# Autodesk Inventor assembly: Gearbox Handle
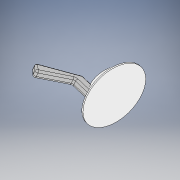
[picture p0: Inventor's stored thumbnail of the model, 180x180]
Saved by Autodesk Inventor 2016 (Build 200138000, 138)
## iProperties
Created: 2017-08-15
Part Number: Gearbox Handle
Document SubType Name: Assembly
Designer: M227562
Author: M227562
## Documents named in this file (3)
- C:\Users\M227562\Documents\My Stuff\Gearbox Stuff\Gearbox Handle.iam
- C:\Users\M227562\Documents\My Stuff\Gearbox Stuff\Handle Gearbox.ipt
- C:\Users\M227562\Documents\My Stuff\Gearbox Stuff\Handle Gearbox handle.ipt
## Components (2 placed, 2 different names)
1. Handle Gearbox:1 — Rigid:1
2. Handle Gearbox handle:1 — Rigid:1
## Relationships (1: WeldJoint 1)
- Rigid:1 [WeldJoint] (-12 mm): Handle Gearbox:1 ↔ Handle Gearbox handle:1
